# Autodesk Inventor assembly: BodyStructure
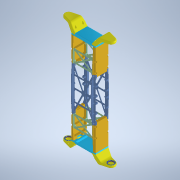
[picture p0: Inventor's stored thumbnail of the model, 180x180]
Saved by Autodesk Inventor 2022.2 (Build 262287000, 287)
## iProperties
Created: 2022-01-14
Part Number: BodyStructure
Document SubType Name: Assembly
Designer: Jochen
Author: Jochen
## Documents named in this file (7)
- D:\Projects\Chewbacca\CAD\BodyStructure.iam
- D:\Projects\Chewbacca\CAD\Body\BodyStructure Side.ipt
- D:\Projects\Chewbacca\CAD\Body\BodyStructure HipSupport.ipt
- D:\Projects\Chewbacca\CAD\Body\BodyStructure Front.ipt
- D:\Projects\Chewbacca\CAD\Body\BodyStructure Centre.ipt
- D:\Projects\Chewbacca\CAD\Body\BodyStructure Plate.ipt
- D:\Projects\Chewbacca\CAD\Common\Bearing\bearing_27_20_4 s61704-2rsr.ipt
## Components (20 placed, 5 different names)
1. BodyStructure Side:1 — Mate:7, Mate:8, Mate:9, Flush:1, Mate:11, Mate:25
2. BodyStructure Side:2 — Mate:5, Mate:6, Mate:30, Mate:32, Mate:33
3. BodyHipSupport:1 — Mate:3, Mate:4, Mate:38, Mate:39
4. BodyHipSupport:2 — Mate:1, Mate:2, Mate:44, Mate:45
5. BodyStructure Front:1 — Mate:1, Mate:2, Mate:3, Mate:4, Mate:5, Mate:6, Mate:7, Mate:8
6. Body Structure Centre:1 — Mate:9, Flush:1, Mate:13, Mate:14, Mate:15, Mate:16, Mate:33, Mate:34, Mate:36
7. Body Structure Centre:2 — Mate:11, Mate:31, Mate:32, Mate:35
8. BodyStructure Side:3 — Mate:13, Mate:16, Mate:20, Mate:28
9. BodyStructure Side:4 — Mate:14, Mate:15, Mate:19, Mate:37
10. BodyStructure Front:2 — Mate:19, Mate:20, Mate:21, Mate:22, Mate:23, Mate:24
11. BodyHipSupport:3 — Mate:23, Mate:24, Mate:42, Mate:43
12. BodyHipSupport:4 — Mate:21, Mate:22, Mate:40, Mate:41
13. Body Structure Centre:3 — Mate:25, Mate:34
14. Body Structure Centre:4 — Mate:28, Mate:36
15. Body Structure Centre:5 — Mate:30, Mate:35
16. Body Structure Centre:6 — Mate:31, Mate:37
17. bearing_27_20_4 s61704-2rsr:1 — Mate:38, Mate:39
18. bearing_27_20_4 s61704-2rsr:2 — Mate:44, Mate:45
19. bearing_27_20_4 s61704-2rsr:3 — Mate:40, Mate:41
20. bearing_27_20_4 s61704-2rsr:4 — Mate:42, Mate:43
## Relationships (39: Mate 38, Flush 1)
- Mate:1: BodyHipSupport:2 ↔ BodyStructure Front:1
- Mate:2: BodyHipSupport:2 ↔ BodyStructure Front:1
- Mate:3: BodyHipSupport:1 ↔ BodyStructure Front:1
- Mate:4: BodyHipSupport:1 ↔ BodyStructure Front:1
- Mate:5: BodyStructure Side:2 ↔ BodyStructure Front:1
- Mate:6: BodyStructure Side:2 ↔ BodyStructure Front:1
- Mate:7: BodyStructure Side:1 ↔ BodyStructure Front:1
- Mate:8: BodyStructure Side:1 ↔ BodyStructure Front:1
- Mate:9: BodyStructure Side:1 ↔ Body Structure Centre:1
- Flush:1: BodyStructure Side:1 ↔ Body Structure Centre:1
- Mate:11: BodyStructure Side:1 ↔ Body Structure Centre:2
- Mate:13: Body Structure Centre:1 ↔ BodyStructure Side:3
- Mate:14: Body Structure Centre:1 ↔ BodyStructure Side:4
- Mate:15: Body Structure Centre:1 ↔ BodyStructure Side:4
- Mate:16: Body Structure Centre:1 ↔ BodyStructure Side:3
- Mate:19: BodyStructure Side:4 ↔ BodyStructure Front:2
- Mate:20: BodyStructure Side:3 ↔ BodyStructure Front:2
- Mate:21: BodyStructure Front:2 ↔ BodyHipSupport:4
- Mate:22: BodyStructure Front:2 ↔ BodyHipSupport:4
- Mate:23: BodyStructure Front:2 ↔ BodyHipSupport:3
- Mate:24: BodyStructure Front:2 ↔ BodyHipSupport:3
- Mate:25: BodyStructure Side:1 ↔ Body Structure Centre:3
- Mate:28: BodyStructure Side:3 ↔ Body Structure Centre:4
- Mate:30: BodyStructure Side:2 ↔ Body Structure Centre:5
- Mate:31: Body Structure Centre:2 ↔ Body Structure Centre:6
- Mate:32: BodyStructure Side:2 ↔ Body Structure Centre:2
- Mate:33: BodyStructure Side:2 ↔ Body Structure Centre:1
- Mate:34: Body Structure Centre:1 ↔ Body Structure Centre:3
- Mate:35: Body Structure Centre:2 ↔ Body Structure Centre:5
- Mate:36: Body Structure Centre:1 ↔ Body Structure Centre:4
- Mate:37: BodyStructure Side:4 ↔ Body Structure Centre:6
- Mate:38: BodyHipSupport:1 ↔ bearing_27_20_4 s61704-2rsr:1
- Mate:39: BodyHipSupport:1 ↔ bearing_27_20_4 s61704-2rsr:1
- Mate:40: BodyHipSupport:4 ↔ bearing_27_20_4 s61704-2rsr:3
- Mate:41: BodyHipSupport:4 ↔ bearing_27_20_4 s61704-2rsr:3
- Mate:42: BodyHipSupport:3 ↔ bearing_27_20_4 s61704-2rsr:4
- Mate:43: BodyHipSupport:3 ↔ bearing_27_20_4 s61704-2rsr:4
- Mate:44: BodyHipSupport:2 ↔ bearing_27_20_4 s61704-2rsr:2
- Mate:45: BodyHipSupport:2 ↔ bearing_27_20_4 s61704-2rsr:2
